# Autodesk Inventor assembly: motor-X83008S
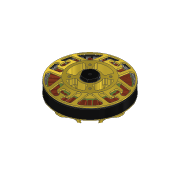
[picture p0: Inventor's stored thumbnail of the model, 180x180]
Saved by Autodesk Inventor 2020 (Build 240168000, 168)
## iProperties
Created: 2020-05-19
Part Number: motor-X83008S
Document SubType Name: Assembly
Designer: Kostic
Author: Kostic
## Documents named in this file (10)
- Z:\Yandex.Disk.localized\Voltbro\xSets\mayatnik\motor-X8308S\motor-X83008S.iam
- Z:\Yandex.Disk.localized\Voltbro\xSets\mayatnik\motor-X8308S\coil.ipt
- Z:\Yandex.Disk.localized\Voltbro\xSets\mayatnik\motor-X8308S\stator.ipt
- Z:\Yandex.Disk.localized\Voltbro\xSets\mayatnik\motor-X8308S\base.ipt
- Z:\Yandex.Disk.localized\Voltbro\xSets\mayatnik\motor-X8308S\rotor.ipt
- Z:\Yandex.Disk.localized\Voltbro\xSets\mayatnik\motor-X8308S\outrunner.ipt
- Z:\Yandex.Disk.localized\Voltbro\xSets\mayatnik\motor-X8308S\screw-mount.ipt
- Z:\Yandex.Disk.localized\Voltbro\xSets\mayatnik\motor-X8308S\6702ZZ-bearing-15x21x4.ipt
- Z:\Yandex.Disk.localized\Voltbro\xSets\mayatnik\motor-X8308S\shaft.ipt
- Z:\Yandex.Disk.localized\Voltbro\xSets\mayatnik\motor-X8308S\fix-screw.ipt
## Components (48 placed, 9 different names)
1. base:1 — Insert:1, Insert:8, Insert:9
2. stator:1 — Mate:1, Mate:2, Mate:3, Insert:1, Insert:2
3. rotor:1 — Insert:2, Insert:3, Mate:4
4. outrunner:1 — Insert:3, Mate:4, Insert:4, Insert:5, Insert:6, Insert:7, Insert:10
5. screw-mount:1 — Insert:4
6. screw-mount:2 — Insert:5
7. screw-mount:3 — Insert:6
8. screw-mount:4 — Insert:7
9. 6702ZZ-bearing-15x21x4:1 — Insert:8, Insert:11
10. 6702ZZ-bearing-15x21x4:2 — Insert:9
11. shaft:1 — Insert:10
12. fix-screw:1 — Insert:11
13. coil:1 — Mate:1, Mate:2, Mate:3
14. coil:2
15. coil:3
16. coil:4
17. coil:5
18. coil:6
19. coil:7
20. coil:8
21. coil:9
22. coil:10
23. coil:11
24. coil:12
25. coil:13
26. coil:14
27. coil:15
28. coil:16
29. coil:17
30. coil:18
31. coil:19
32. coil:20
33. coil:21
34. coil:22
35. coil:23
36. coil:24
37. coil:25
38. coil:26
39. coil:27
40. coil:28
41. coil:29
42. coil:30
43. coil:31
44. coil:32
45. coil:33
46. coil:34
47. coil:35
48. coil:36
## Component patterns: (36 elements, first: coil:1)
## Relationships (15: Insert 11, Mate 4)
- Mate:1: stator:1 ↔ coil:1
- Mate:2: stator:1 ↔ coil:1
- Mate:3: stator:1 ↔ coil:1
- Insert:1: base:1 ↔ stator:1
- Insert:2 (-3 mm): stator:1 ↔ rotor:1
- Insert:3: rotor:1 ↔ outrunner:1
- Mate:4: rotor:1 ↔ outrunner:1
- Insert:4: outrunner:1 ↔ screw-mount:1
- Insert:5: outrunner:1 ↔ screw-mount:2
- Insert:6: outrunner:1 ↔ screw-mount:3
- Insert:7: outrunner:1 ↔ screw-mount:4
- Insert:8: base:1 ↔ 6702ZZ-bearing-15x21x4:1
- Insert:9: base:1 ↔ 6702ZZ-bearing-15x21x4:2
- Insert:10: outrunner:1 ↔ shaft:1
- Insert:11: 6702ZZ-bearing-15x21x4:1 ↔ fix-screw:1
